# Autodesk Inventor assembly: #Turret
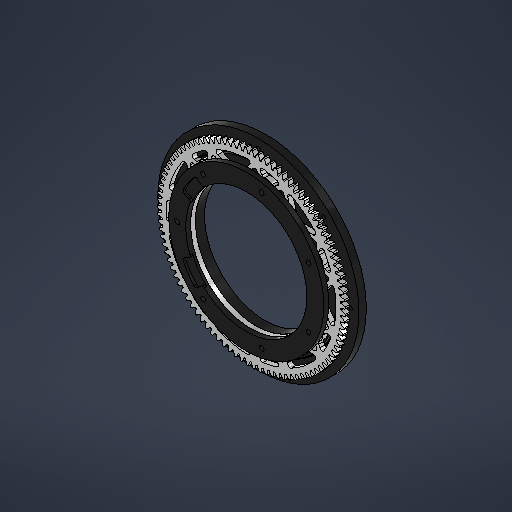
[picture p0: Inventor's stored thumbnail of the model, 512x512]
Saved by Autodesk Inventor 2026 (Build 300175000, 175)
## iProperties
Created: 2026-02-01
Part Number: #Turret
Document SubType Name: Assembly
Designer: Owen L
Mass: 706.354 g
Surface Area: 1883.53 cm^2
Volume: 481.196 cm^3
Density: 1.46791 g/cm^3
Author: Owen L
## Documents named in this file (5)
- C:\Users\littl\OneDrive\Documents\GitHub\2026-Robot-Mechanical\Shooter\Turret\#Turret.iam
- C:\Users\littl\OneDrive\Documents\GitHub\2026-Robot-Mechanical\Shooter\Turret\3DPRINT,TURRET,BEARING,INNER.ipt
- C:\Users\littl\OneDrive\Documents\GitHub\2026-Robot-Mechanical\Shooter\Turret\3DPRINT,TURRET,BEARING,OUTER.ipt
- C:\Users\littl\OneDrive\Documents\GitHub\2026-Robot-Mechanical\Shooter\Turret\#Turret\Design Accelerator\PLATE,TURRET,GEAR.ipt
- C:\Users\littl\OneDrive\Documents\GitHub\2026-Robot-Mechanical\Shooter\Turret\3DPRINT,TURRET,SPACER.ipt
## Components (4 placed, 4 different names)
1. 3DPRINT,TURRET,BEARING,INNER:1 — Flush:1, Mate:1, Mate:2, Mate:3, Mate:4
2. 3DPRINT,TURRET,BEARING,OUTER:1 — Flush:1, Mate:1
3. PLATE,TURRET,GEAR:1 — Mate:2, Mate:3, Mate:4, Mate:5, Mate:6, Mate:7
4. 3DPRINT,TURRET,SPACER:1 — Mate:5, Mate:6, Mate:7
## Relationships (8: Mate 7, Flush 1)
- Flush:1 (-0.7937 mm): 3DPRINT,TURRET,BEARING,INNER:1 ↔ 3DPRINT,TURRET,BEARING,OUTER:1
- Mate:1: 3DPRINT,TURRET,BEARING,INNER:1 ↔ 3DPRINT,TURRET,BEARING,OUTER:1
- Mate:2: 3DPRINT,TURRET,BEARING,INNER:1 ↔ PLATE,TURRET,GEAR:1
- Mate:3: 3DPRINT,TURRET,BEARING,INNER:1 ↔ PLATE,TURRET,GEAR:1
- Mate:4: 3DPRINT,TURRET,BEARING,INNER:1 ↔ PLATE,TURRET,GEAR:1
- Mate:5: PLATE,TURRET,GEAR:1 ↔ 3DPRINT,TURRET,SPACER:1
- Mate:6: PLATE,TURRET,GEAR:1 ↔ 3DPRINT,TURRET,SPACER:1
- Mate:7: PLATE,TURRET,GEAR:1 ↔ 3DPRINT,TURRET,SPACER:1
